# Autodesk Inventor assembly: wheel_axle
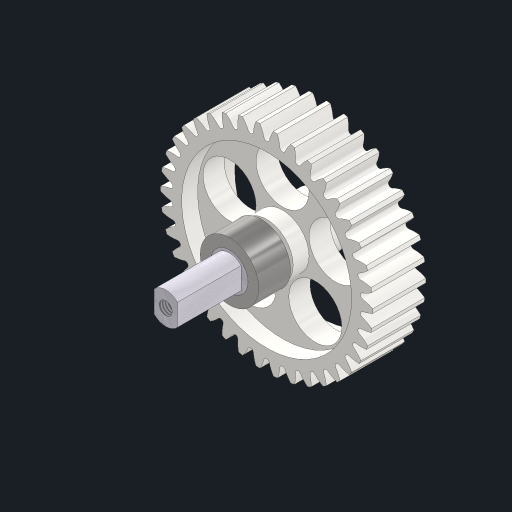
[picture p0: Inventor's stored thumbnail of the model, 512x512]
Saved by Autodesk Inventor 2023 (Build 270158000, 158)
## iProperties
Created: 2024-04-09
Part Number: wheel_axle
Document SubType Name: Assembly
Designer: szymo
Mass: 30 g
Surface Area: 69.3563 cm^2
Volume: 6.5273 cm^3
Density: 4.59608 g/cm^3
Author: szymo
## Documents named in this file (5)
- C:\zRozne\roboilo\robots\wafel\3d_parts\wheel_axle.iam
- C:\zRozne\roboilo\robots\wafel\3d_parts\MegaSumo kola zebate 38.ipt
- C:\zRozne\roboilo\robots\wafel\3d_parts\wal_kola.ipt
- C:\zRozne\roboilo\robots\wafel\3d_parts\small_bearing.ipt
- C:\zRozne\roboilo\robots\wafel\3d_parts\big_bearing.ipt
## Components (4 placed, 4 different names)
1. wal_kola:1 — Rotational:1, Flush:1, Flush:2
2. MegaSumo kola zebate 38:1 — Rotational:1
3. small_bearing:1 — Flush:1
4. big_bearing:1 — Flush:2
## Relationships (3: Flush 2, RevoluteJoint 1)
- Rotational:1 [RevoluteJoint]: wal_kola:1 ↔ MegaSumo kola zebate 38:1
- Flush:1: wal_kola:1 ↔ small_bearing:1
- Flush:2: wal_kola:1 ↔ big_bearing:1
